# Autodesk Inventor assembly: zlozeniedrona
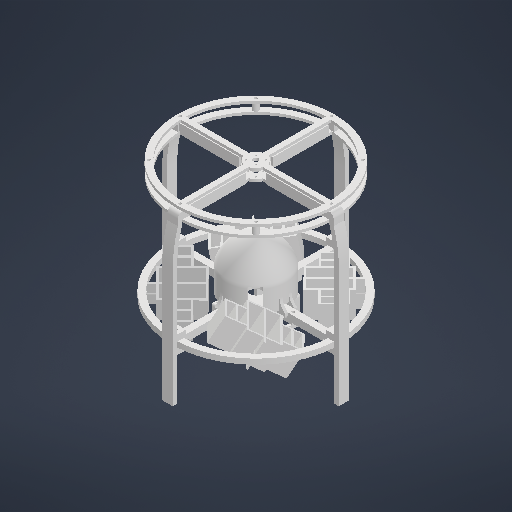
[picture p0: Inventor's stored thumbnail of the model, 512x512]
Saved by Autodesk Inventor 2026.2 (Build 302298010, 298A)
## iProperties
Created: 2026-04-18
Part Number: zlozeniedrona
Document SubType Name: Assembly
Designer: macie
Author: macie
## Documents named in this file (9)
- C:\Users\macie\Documents\dron\zlozeniedrona.iam
- C:\Users\macie\Documents\dron\rama-silnik-dol-2.ipt
- C:\Users\macie\Documents\dron\rama-silnik-gora-1.ipt
- C:\Users\macie\Documents\dron\mocowanie-serwomechanizmy.ipt
- C:\Users\macie\Documents\dron\podstawa-serwomechanizmy.ipt
- C:\Users\macie\Documents\dron\pokrywa-podstawy.ipt
- C:\Users\macie\Documents\dron\podpory.ipt
- C:\Users\macie\Documents\dron\mocowanie-controller.ipt
- C:\Users\macie\Documents\dron\klapy.ipt
## Components (17 placed, 8 different names)
1. rama-silnik-dol-2:1 — Obrotowe:1, Zestawiające:1, Wstawiające:11, Zestawiające:2, Wstawiające:12, Wstawiające:13, Styczny:1, Styczny:2, Styczny:3, Wstawiające:15, Styczny:4
2. rama-silnik-gora-1:1 — Obrotowe:1, Zestawiające:1
3. podstawa-serwomechanizmy:1 — Wstawiające:1, Wstawiające:2, Wstawiające:3, Wstawiające:4, Wstawiające:5, Wstawiające:6, Wstawiające:7, Wstawiające:8, Wstawiające:9, Wstawiające:10, Wstawiające:14, Styczny:5, Wstawiające:16, Wstawiające:17, Obrotowe:2, Obrotowe:3, Obrotowe:4, Obrotowe:5
4. mocowanie-serwomechanizmy:2 — Wstawiające:7, Wstawiające:8
5. mocowanie-serwomechanizmy:3 — Wstawiające:5, Wstawiające:6
6. mocowanie-serwomechanizmy:4 — Wstawiające:3, Wstawiające:4
7. mocowanie-serwomechanizmy:5 — Wstawiające:1, Wstawiające:2
8. pokrywa-podstawy:1 — Wstawiające:9, Wstawiające:10
9. podpory:1 — Wstawiające:11, Styczny:3, Styczny:5
10. podpory:2 — Zestawiające:2, Wstawiające:15, Styczny:4
11. podpory:3 — Wstawiające:12, Wstawiające:14, Styczny:1
12. podpory:4 — Wstawiające:13, Styczny:2
13. mocowanie-controller:1 — Wstawiające:16, Wstawiające:17
14. klapy:1 — Obrotowe:2
15. klapy:2 — Obrotowe:3
16. klapy:3 — Obrotowe:4
17. klapy:4 — Obrotowe:5
## Relationships (29: Insert 17, RevoluteJoint 5, Tangent 5, Mate 2)
- Obrotowe:1 [RevoluteJoint]: rama-silnik-dol-2:1 ↔ rama-silnik-gora-1:1
- Zestawiające:1 [Mate]: rama-silnik-dol-2:1 ↔ rama-silnik-gora-1:1
- Wstawiające:1 [Insert]: podstawa-serwomechanizmy:1 ↔ mocowanie-serwomechanizmy:5
- Wstawiające:2 [Insert]: podstawa-serwomechanizmy:1 ↔ mocowanie-serwomechanizmy:5
- Wstawiające:3 [Insert]: podstawa-serwomechanizmy:1 ↔ mocowanie-serwomechanizmy:4
- Wstawiające:4 [Insert]: podstawa-serwomechanizmy:1 ↔ mocowanie-serwomechanizmy:4
- Wstawiające:5 [Insert]: podstawa-serwomechanizmy:1 ↔ mocowanie-serwomechanizmy:3
- Wstawiające:6 [Insert]: podstawa-serwomechanizmy:1 ↔ mocowanie-serwomechanizmy:3
- Wstawiające:7 [Insert]: podstawa-serwomechanizmy:1 ↔ mocowanie-serwomechanizmy:2
- Wstawiające:8 [Insert]: podstawa-serwomechanizmy:1 ↔ mocowanie-serwomechanizmy:2
- Wstawiające:9 [Insert]: podstawa-serwomechanizmy:1 ↔ pokrywa-podstawy:1
- Wstawiające:10 [Insert]: podstawa-serwomechanizmy:1 ↔ pokrywa-podstawy:1
- Wstawiające:11 [Insert]: rama-silnik-dol-2:1 ↔ podpory:1
- Zestawiające:2 [Mate]: rama-silnik-dol-2:1 ↔ podpory:2
- Wstawiające:12 [Insert]: rama-silnik-dol-2:1 ↔ podpory:3
- Wstawiające:13 [Insert]: rama-silnik-dol-2:1 ↔ podpory:4
- Wstawiające:14 [Insert]: podstawa-serwomechanizmy:1 ↔ podpory:3
- Styczny:1 [Tangent]: rama-silnik-dol-2:1 ↔ podpory:3
- Styczny:2 [Tangent]: rama-silnik-dol-2:1 ↔ podpory:4
- Styczny:3 [Tangent]: rama-silnik-dol-2:1 ↔ podpory:1
- Wstawiające:15 [Insert]: rama-silnik-dol-2:1 ↔ podpory:2
- Styczny:4 [Tangent]: rama-silnik-dol-2:1 ↔ podpory:2
- Styczny:5 [Tangent]: podstawa-serwomechanizmy:1 ↔ podpory:1
- Wstawiające:16 [Insert]: podstawa-serwomechanizmy:1 ↔ mocowanie-controller:1
- Wstawiające:17 [Insert]: podstawa-serwomechanizmy:1 ↔ mocowanie-controller:1
- Obrotowe:2 [RevoluteJoint]: podstawa-serwomechanizmy:1 ↔ klapy:1
- Obrotowe:3 [RevoluteJoint]: podstawa-serwomechanizmy:1 ↔ klapy:2
- Obrotowe:4 [RevoluteJoint]: podstawa-serwomechanizmy:1 ↔ klapy:3
- Obrotowe:5 [RevoluteJoint]: podstawa-serwomechanizmy:1 ↔ klapy:4
